# Autodesk Inventor assembly: Assembly1
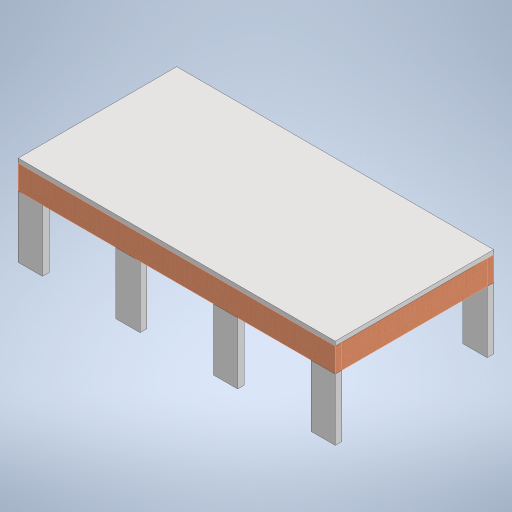
[picture p0: Inventor's stored thumbnail of the model, 512x512]
Saved by Autodesk Inventor 2023 (Build 270158000, 158)
## iProperties
Created: 2022-08-19
Part Number: Assembly1
Document SubType Name: Assembly
Designer: rkant
Mass: 16189.9 g
Surface Area: 19393.5 cm^2
Volume: 28390.6 cm^3
Density: 0.570257 g/cm^3
Author: rkant
## Documents named in this file (6)
- C:\Users\rkant\Desktop\Inventor\Stock Holder\Assembly1.iam
- C:\Users\rkant\Desktop\Inventor\Stock Holder\2x6x6'.ipt
- C:\Users\rkant\Desktop\Inventor\Stock Holder\2x6x3'.ipt
- C:\Users\rkant\Desktop\Inventor\Stock Holder\6'x3' plywood.ipt
- C:\Users\rkant\Desktop\Inventor\Stock Holder\legs.ipt
- C:\Users\rkant\Desktop\Inventor\Stock Holder\legs_MIR.ipt
## Components (15 placed, 5 different names)
1. 2x6x6':1 — Mate:1, Mate:2, Flush:3, Flush:4, Mate:6, Flush:5, Mate:7, Flush:7, Flush:8
2. 2x6x6':2 — Mate:1, Mate:2, Mate:3, Flush:1, Mate:4, Flush:2, Mate:5
3. 2x6x3':1 — Mate:3, Flush:1, Mate:4, Flush:2, Flush:6
4. 6'x3' plywood:2 — Mate:6, Flush:5, Flush:6
5. legs_MIR:1
6. legs_MIR:2
7. legs_MIR:3
8. legs_MIR:4
9. legs:1 — Mate:7, Flush:7, Flush:8
10. legs:2
11. legs:3
12. legs:4
13. 2x6x3':2 — Mate:5, Flush:3, Flush:4
14. 2x6x3':3
15. 2x6x3':4
## Component patterns: (4 elements, first: legs:1), (3 elements, first: 2x6x3':2)
## Relationships (15: Flush 8, Mate 7)
- Mate:1 (914.4 mm): 2x6x6':1 ↔ 2x6x6':2
- Mate:2: 2x6x6':1 ↔ 2x6x6':2
- Mate:3: 2x6x6':2 ↔ 2x6x3':1
- Flush:1: 2x6x6':2 ↔ 2x6x3':1
- Mate:4: 2x6x6':2 ↔ 2x6x3':1
- Flush:2: 2x6x6':2 ↔ 2x6x3':1
- Mate:5: 2x6x6':2 ↔ 2x6x3':2
- Flush:3: 2x6x6':1 ↔ 2x6x3':2
- Flush:4: 2x6x6':1 ↔ 2x6x3':2
- Mate:6: 2x6x6':1 ↔ 6'x3' plywood:2
- Flush:5: 2x6x6':1 ↔ 6'x3' plywood:2
- Flush:6: 2x6x3':1 ↔ 6'x3' plywood:2
- Mate:7: 2x6x6':1 ↔ legs:1
- Flush:7: 2x6x6':1 ↔ legs:1
- Flush:8: 2x6x6':1 ↔ legs:1
